# Autodesk Inventor assembly: Assemble
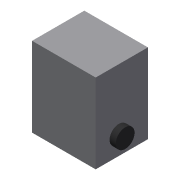
[picture p0: Inventor's stored thumbnail of the model, 180x180]
Saved by Autodesk Inventor 2019 (Build 230136000, 136)
## iProperties
Created: 2019-04-28
Part Number: Assemble
Material: 일반
Document SubType Name: Assembly
Designer: hinmo
Author: hinmo
## Documents named in this file (3)
- C:\Users\hinmo\Documents\Inventor\Projects\2019_CapstoneDesignSimple\Assemble.iam
- C:\Users\hinmo\Documents\Inventor\Projects\2019_CapstoneDesignSimple\Body.ipt
- C:\Users\hinmo\Documents\Inventor\Projects\2019_CapstoneDesignSimple\Wheel.ipt
## Components (3 placed, 2 different names)
1. Body:1 — 메이트:1, 메이트:2, 메이트:3, 메이트:5, 메이트:6
2. Wheel:1 — 메이트:4, 메이트:6
3. Wheel:2 — 메이트:4, 메이트:5
## Relationships (6: Mate 6)
- 메이트:1 [Mate]: Body:1
- 메이트:2 [Mate]: Body:1
- 메이트:3 [Mate]: Body:1
- 메이트:4 [Mate]: Wheel:1 ↔ Wheel:2
- 메이트:5 [Mate]: Body:1 ↔ Wheel:2
- 메이트:6 [Mate]: Body:1 ↔ Wheel:1
